# Autodesk Inventor assembly: FactionTray
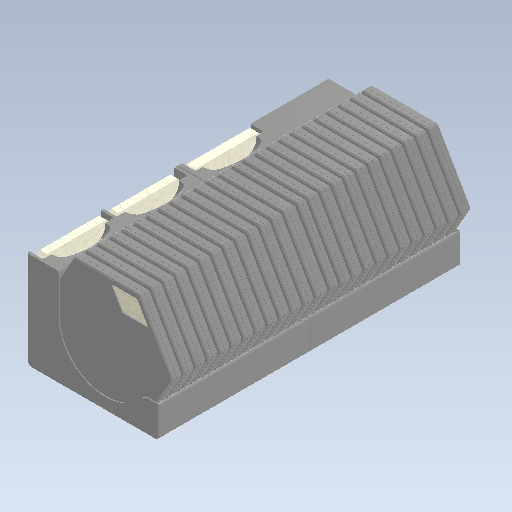
[picture p0: Inventor's stored thumbnail of the model, 512x512]
Saved by Autodesk Inventor 2021 (Build 250183000, 183)
## iProperties
Created: 2023-03-17
Part Number: FactionTray
Document SubType Name: Assembly
Designer: Bradley
Author: Bradley
## Documents named in this file (9)
- C:\Users\Bradley\Git\TI4\Factions\FactionTray.iam
- C:\Users\Bradley\Git\TI4\Factions\FactionTray_B.ipt
- C:\Users\Bradley\Git\TI4\Factions\FactionTray_A.ipt
- C:\Users\Bradley\Git\TI4\Factions\FactionTray_Pin.ipt
- C:\Users\Bradley\Git\TI4\Factions\Factions_Normal.iam
- C:\Users\Bradley\Git\TI4\Factions\Factions_Council.iam
- C:\Users\Bradley\Git\TI4\Factions\Factions_Embers.iam
- C:\Users\Bradley\Git\TI4\Components\StrategyCard_Single.ipt
- C:\Users\Bradley\Git\TI4\Components\FactionReference_All.ipt
## Components (39 placed, 8 different names)
1. FactionTray_B:1 — Insert:1, Insert:2, Insert:3, Insert:4, Insert:5, Mate:1, Mate:2, Mate:3, Mate:4, Mate:16, Mate:17, Mate:18, Mate:22, Mate:23
2. FactionTray_A:1 — Insert:4, Insert:5, Mate:5, Mate:6, Mate:7, Mate:8, Mate:9, Mate:10, Mate:11, Mate:12, Mate:24, Mate:25, Mate:26
3. FactionTray_Pin:1 — Insert:3
4. FactionTray_Pin:2 — Insert:2
5. FactionTray_Pin:3 — Insert:1
6. Factions_Council:1 [sub-assembly] — Mate:7, Mate:8, Mate:9
7. Factions_Embers:1 [sub-assembly] — Mate:4, Mate:5, Mate:6
8. StrategyCard_Single:1 — Mate:13, Flush:1, Flush:4, Mate:16, Mate:17, Mate:18
9. StrategyCard_Single:2 — Mate:13, Mate:14, Flush:1, Flush:2, Flush:4, Flush:5
10. StrategyCard_Single:3 — Mate:14, Mate:15, Flush:2, Flush:3, Flush:5, Flush:6
11. StrategyCard_Single:4 — Mate:15, Flush:3, Flush:6, Flush:13
12. StrategyCard_Single:5 — Mate:22, Mate:23, Flush:13
13. StrategyCard_Single:6
14. StrategyCard_Single:7
15. StrategyCard_Single:8
16. FactionReference_All:1 — Mate:24, Mate:25, Mate:26
17. Factions_Normal:1 [sub-assembly] — Mate:1, Mate:2, Mate:3
18. Factions_Normal:3 [sub-assembly]
19. Factions_Normal:4 [sub-assembly]
20. Factions_Normal:5 [sub-assembly]
21. Factions_Normal:6 [sub-assembly]
22. Factions_Normal:7 [sub-assembly]
23. Factions_Normal:8 [sub-assembly]
24. Factions_Normal:9 [sub-assembly]
25. Factions_Normal:10 [sub-assembly]
26. Factions_Normal:11 [sub-assembly]
27. Factions_Normal:12 [sub-assembly]
28. Factions_Normal:13 [sub-assembly]
29. Factions_Normal:2 [sub-assembly] — Mate:10, Mate:11, Mate:12
30. Factions_Normal:14 [sub-assembly]
31. Factions_Normal:15 [sub-assembly]
32. Factions_Normal:16 [sub-assembly]
33. Factions_Normal:17 [sub-assembly]
34. Factions_Normal:18 [sub-assembly]
35. Factions_Normal:19 [sub-assembly]
36. Factions_Normal:20 [sub-assembly]
37. Factions_Normal:21 [sub-assembly]
38. Factions_Normal:22 [sub-assembly]
39. Factions_Normal:23 [sub-assembly]
## Component patterns: (12 elements, first: Factions_Normal:1), (11 elements, first: Factions_Normal:2)
## Relationships (44: Mate 26, Flush 13, Insert 5)
- Insert:1: FactionTray_B:1 ↔ FactionTray_Pin:3
- Insert:2: FactionTray_B:1 ↔ FactionTray_Pin:2
- Insert:3: FactionTray_B:1 ↔ FactionTray_Pin:1
- Insert:4: FactionTray_B:1 ↔ FactionTray_A:1
- Insert:5: FactionTray_B:1 ↔ FactionTray_A:1
- Mate:1 (0.322 mm): FactionTray_B:1 ↔ Factions_Normal:1
- Mate:2: FactionTray_B:1 ↔ Factions_Normal:1
- Mate:3 (0.25 mm): FactionTray_B:1 ↔ Factions_Normal:1
- Mate:4 (0.322 mm): FactionTray_B:1 ↔ Factions_Embers:1
- Mate:5: FactionTray_A:1 ↔ Factions_Embers:1
- Mate:6 (0.25 mm): FactionTray_A:1 ↔ Factions_Embers:1
- Mate:7 (0.322 mm): FactionTray_A:1 ↔ Factions_Council:1
- Mate:8: FactionTray_A:1 ↔ Factions_Council:1
- Mate:9 (0.25 mm): FactionTray_A:1 ↔ Factions_Council:1
- Mate:10 (0.322 mm): FactionTray_A:1 ↔ Factions_Normal:2
- Mate:11: FactionTray_A:1 ↔ Factions_Normal:2
- Mate:12 (0.25 mm): FactionTray_A:1 ↔ Factions_Normal:2
- Mate:13: StrategyCard_Single:1 ↔ StrategyCard_Single:2
- Mate:14: StrategyCard_Single:2 ↔ StrategyCard_Single:3
- Mate:15: StrategyCard_Single:3 ↔ StrategyCard_Single:4
- Flush:1: StrategyCard_Single:1 ↔ StrategyCard_Single:2
- Flush:2: StrategyCard_Single:2 ↔ StrategyCard_Single:3
- Flush:3: StrategyCard_Single:3 ↔ StrategyCard_Single:4
- Flush:4: StrategyCard_Single:1 ↔ StrategyCard_Single:2
- Flush:5: StrategyCard_Single:2 ↔ StrategyCard_Single:3
- Flush:6: StrategyCard_Single:3 ↔ StrategyCard_Single:4
- Mate:16: FactionTray_B:1 ↔ StrategyCard_Single:1
- Mate:17 (1 mm): FactionTray_B:1 ↔ StrategyCard_Single:1
- Mate:18 (0.5 mm): FactionTray_B:1 ↔ StrategyCard_Single:1
- [Mate]: StrategyCard_Single:5 ↔ StrategyCard_Single:6
- [Mate]: StrategyCard_Single:6 ↔ StrategyCard_Single:7
- [Mate]: StrategyCard_Single:7 ↔ StrategyCard_Single:8
- [Flush]: StrategyCard_Single:5 ↔ StrategyCard_Single:6
- [Flush]: StrategyCard_Single:6 ↔ StrategyCard_Single:7
- [Flush]: StrategyCard_Single:7 ↔ StrategyCard_Single:8
- [Flush]: StrategyCard_Single:5 ↔ StrategyCard_Single:6
- [Flush]: StrategyCard_Single:6 ↔ StrategyCard_Single:7
- [Flush]: StrategyCard_Single:7 ↔ StrategyCard_Single:8
- Mate:22: FactionTray_B:1 ↔ StrategyCard_Single:5
- Mate:23 (0.5 mm): FactionTray_B:1 ↔ StrategyCard_Single:5
- Flush:13: StrategyCard_Single:4 ↔ StrategyCard_Single:5
- Mate:24 (0.4 mm): FactionTray_A:1 ↔ FactionReference_All:1
- Mate:25 (0.5 mm): FactionTray_A:1 ↔ FactionReference_All:1
- Mate:26: FactionTray_A:1 ↔ FactionReference_All:1
## Named parameters: PuckGap = 0.644 mm, PuckNormalSpacing = 11.344 mm, d37_d25 = 0 mm, d38_d26 = 0 mm, d39_d27 = 0 mm, d40_d28 = 0 mm, d41_d29 = 0 mm, d42_d30 = 0 mm, d43_d31 = 0 mm, d44_d32 = 0 mm, d45_d33 = 0 mm
